# Autodesk Inventor assembly: Assembly Plate with Cover
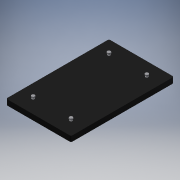
[picture p0: Inventor's stored thumbnail of the model, 180x180]
Saved by Autodesk Inventor 2019.4 (Build 234330000, 330)
## iProperties
Created: 2021-01-28
Part Number: Assembly Plate with Cover
Document SubType Name: Assembly
Designer: caleb
Author: caleb
## Documents named in this file (4)
- C:\Users\cfang\Desktop\nebraska-silicon-lab\CAD\ETL\Module Assembly\Assembly Plate\Assembly Plate with Cover.iam
- C:\Users\cfang\Desktop\nebraska-silicon-lab\CAD\ETL\Module Assembly\Assembly Plate\Assembly Plate Assembly.iam
- C:\Users\cfang\Desktop\nebraska-silicon-lab\CAD\ETL\Module Assembly\Assembly Plate\Cover.ipt
- C:\Users\cfang\Desktop\nebraska-silicon-lab\CAD\ETL\Module Assembly\Assembly Plate\99607A272_SS FLARED-COLLAR KNURLED-HEAD THUMB SCREW.ipt
## Components (6 placed, 3 different names)
1. Assembly Plate Assembly:1 [sub-assembly] — Mate:1, Angle:1, Insert:1
2. Cover:1 — Mate:1, Angle:1, Insert:1, Insert:2, Insert:3, Insert:4, Insert:5
3. 99607A272_SS FLARED-COLLAR KNURLED-HEAD THUMB SCREW:1 — Insert:2
4. 99607A272_SS FLARED-COLLAR KNURLED-HEAD THUMB SCREW:2 — Insert:3
5. 99607A272_SS FLARED-COLLAR KNURLED-HEAD THUMB SCREW:3 — Insert:4
6. 99607A272_SS FLARED-COLLAR KNURLED-HEAD THUMB SCREW:4 — Insert:5
## Relationships (7: Insert 5, Mate 1, Angle 1)
- Mate:1: Assembly Plate Assembly:1 ↔ Cover:1
- Angle:1 (0 deg): Assembly Plate Assembly:1 ↔ Cover:1
- Insert:1: Assembly Plate Assembly:1 ↔ Cover:1
- Insert:2: Cover:1 ↔ 99607A272_SS FLARED-COLLAR KNURLED-HEAD THUMB SCREW:1
- Insert:3: Cover:1 ↔ 99607A272_SS FLARED-COLLAR KNURLED-HEAD THUMB SCREW:2
- Insert:4: Cover:1 ↔ 99607A272_SS FLARED-COLLAR KNURLED-HEAD THUMB SCREW:3
- Insert:5: Cover:1 ↔ 99607A272_SS FLARED-COLLAR KNURLED-HEAD THUMB SCREW:4
